# Autodesk Inventor assembly: Montagem
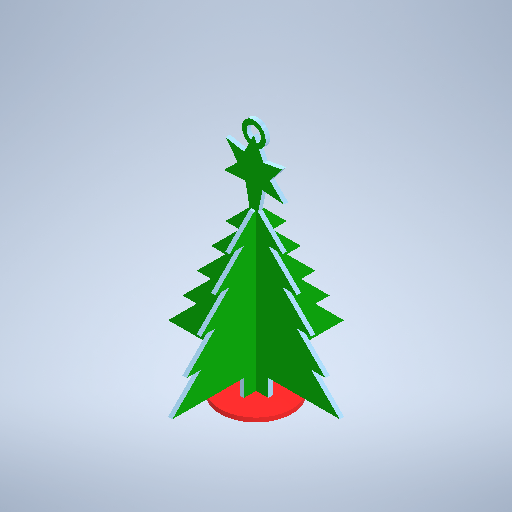
[picture p0: Inventor's stored thumbnail of the model, 512x512]
Saved by Autodesk Inventor 2025 (Build 290162000, 162)
## iProperties
Created: 2024-12-03
Part Number: Montagem
Document SubType Name: Assembly
Designer: Inteli
Author: Inteli
## Documents named in this file (4)
- C:\Users\Inteli\Desktop\Montagem.iam
- C:\Users\Inteli\Desktop\part 1 arvore de natal.ipt
- C:\Users\Inteli\Desktop\part 2 arvore de natal.ipt
- C:\Users\Inteli\Desktop\Base Arvore.ipt
## Components (3 placed, 3 different names)
1. part 1 arvore de natal:1 — Mate:1, Mate:2, Mate:3, Mate:5
2. part 2 arvore de natal:1 — Mate:1, Mate:2, Mate:3, Flush:1, Mate:4
3. Base Arvore:1 — Flush:1, Mate:4, Mate:5
## Relationships (6: Mate 5, Flush 1)
- Mate:1: part 1 arvore de natal:1 ↔ part 2 arvore de natal:1
- Mate:2: part 1 arvore de natal:1 ↔ part 2 arvore de natal:1
- Mate:3: part 1 arvore de natal:1 ↔ part 2 arvore de natal:1
- Flush:1: part 2 arvore de natal:1 ↔ Base Arvore:1
- Mate:4: part 2 arvore de natal:1 ↔ Base Arvore:1
- Mate:5: part 1 arvore de natal:1 ↔ Base Arvore:1
